# Autodesk Inventor assembly: Support
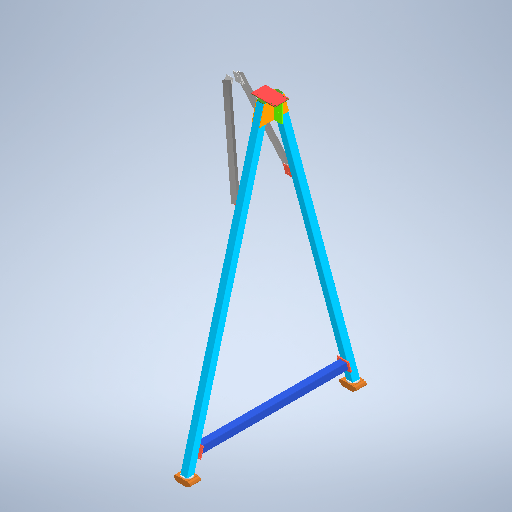
[picture p0: Inventor's stored thumbnail of the model, 512x512]
Saved by Autodesk Inventor 2025 (Build 290162010, 162A)
## iProperties
Created: 2024-06-18
Part Number: Support
Document SubType Name: Assembly
Designer: admin
Stock Number: Опора
Author: admin
## Documents named in this file (13)
- C:\Users\pokla\Documents\Inventor\Goat\Support.iam
- C:\Users\pokla\Documents\Inventor\Goat\Сrane plate 3.ipt
- C:\Users\pokla\Documents\Inventor\Goat\Stand.ipt
- C:\Users\pokla\Documents\Inventor\Goat\Сrane plate 4.ipt
- C:\Users\pokla\Documents\Inventor\Goat\Сrane plate 6.ipt
- C:\Users\pokla\Documents\Inventor\Goat\Сrane plate 2.ipt
- C:\Users\pokla\Documents\Inventor\Goat\Сrane plate 5.ipt
- C:\Users\pokla\Documents\Inventor\Goat\roller platform.ipt
- C:\Users\pokla\Documents\Inventor\Goat\foot.ipt
- C:\Users\pokla\Documents\Inventor\Goat\Crossbar.ipt
- C:\Users\pokla\Documents\Inventor\Goat\Сrane plate 1.ipt
- C:\Users\pokla\Documents\Inventor\Goat\Оттяжки.iam
- C:\Users\pokla\Documents\Inventor\Goat\Оттяжка 2.iam
## Components (24 placed, 12 different names)
1. Сrane plate 3.ipt:1 — Mate:11, Mate:12, Mate:13, Flush:6, Flush:7, Rigid:3
2. Stand.ipt:1 — Mate:9, Mate:10, Rigid:1
3. Сrane plate 4.ipt:1
4. Сrane plate 6.ipt:1 — Rigid:7
5. Сrane plate 4.ipt:2
6. Сrane plate 2.ipt:1 — Mate:11, Mate:12, Mate:13
7. Сrane plate 5.ipt:1 — Mate:9, Mate:10
8. roller platform.ipt:1 — Rigid:2, Mate:14
9. foot.ipt:1 — Rigid:1, Rigid:2
10. Сrane plate 3.ipt:2 — Rigid:3, Rigid:4, Mate:18, Mate:20
11. Сrane plate 2.ipt:2 — Rigid:4, Mate:19, Mate:21, Mate:23, Rigid:9
12. Сrane plate 4.ipt:3 — Mate:18, Mate:19, Flush:12, Flush:13
13. Сrane plate 4.ipt:4 — Mate:20, Mate:21, Mate:22, Mate:24
14. Stand.ipt:2 — Mate:23, Mate:24, Flush:13, Rigid:5, Mate:26, Mate:29, Flush:31, Mate:35, Mate:38
15. foot.ipt:2 — Rigid:5, Rigid:6
16. roller platform.ipt:2 — Rigid:6
17. Сrane plate 6.ipt:2 — Mate:26, Mate:27, Rigid:8, Mate:38
18. Сrane plate 5.ipt:3 — Mate:29, Flush:31, Mate:35
19. Сrane plate 6.ipt:3 — Rigid:7
20. Сrane plate 6.ipt:4 — Rigid:8, Mate:41
21. Crossbar.ipt:1 — Mate:39, Mate:40, Mate:41
22. Сrane plate 1:1 — Rigid:9
23. Оттяжки:1 [sub-assembly]
24. Оттяжка 2:1 [sub-assembly]
## Relationships (52: Mate 31, Flush 10, WeldJoint 9, RevoluteJoint 2)
- [Mate]: Stand.ipt:1 ↔ Сrane plate 4.ipt:1
- [Mate]: Stand.ipt:1 ↔ Сrane plate 4.ipt:2
- [Flush]: Stand.ipt:1 ↔ Сrane plate 4.ipt:2
- [Flush]: Stand.ipt:1 ↔ Сrane plate 4.ipt:1
- [Flush]: Stand.ipt:1 ↔ Сrane plate 4.ipt:1
- [Flush]: Stand.ipt:1 ↔ Сrane plate 4.ipt:2
- [Flush]: Stand.ipt:1 ↔ Сrane plate 2.ipt:1
- [Mate]: Stand.ipt:1 ↔ Сrane plate 2.ipt:1
- [Mate]: Stand.ipt:1 ↔ Сrane plate 6.ipt:1
- [Mate]: Stand.ipt:1 ↔ Сrane plate 6.ipt:1
- [Mate]: Сrane plate 3.ipt:1 ↔ Сrane plate 4.ipt:2
- [Mate] (-200 mm): Stand.ipt:1 ↔ Сrane plate 6.ipt:1
- [Mate]: Stand.ipt:1 ↔ Сrane plate 5.ipt:1
- Mate:9 (-45 mm): Stand.ipt:1 ↔ Сrane plate 5.ipt:1
- Mate:10 (1271 mm): Stand.ipt:1 ↔ Сrane plate 5.ipt:1
- Mate:11: Сrane plate 3.ipt:1 ↔ Сrane plate 2.ipt:1
- Mate:12: Сrane plate 3.ipt:1 ↔ Сrane plate 2.ipt:1
- Mate:13: Сrane plate 3.ipt:1 ↔ Сrane plate 2.ipt:1
- Flush:6: Сrane plate 3.ipt:1
- Flush:7: Сrane plate 3.ipt:1
- Rigid:1 [WeldJoint]: Stand.ipt:1 ↔ foot.ipt:1
- Rigid:2 [WeldJoint]: roller platform.ipt:1 ↔ foot.ipt:1
- Mate:14: roller platform.ipt:1
- [RevoluteJoint]: Сrane plate 5.ipt:1 ↔ Оттяжки:1
- Rigid:3 [WeldJoint]: Сrane plate 3.ipt:1 ↔ Сrane plate 3.ipt:2
- Rigid:4 [WeldJoint]: Сrane plate 3.ipt:2 ↔ Сrane plate 2.ipt:2
- Mate:18: Сrane plate 3.ipt:2 ↔ Сrane plate 4.ipt:3
- Mate:19: Сrane plate 2.ipt:2 ↔ Сrane plate 4.ipt:3
- Flush:12 (60 mm): Сrane plate 4.ipt:3
- Mate:20: Сrane plate 3.ipt:2 ↔ Сrane plate 4.ipt:4
- Mate:21: Сrane plate 2.ipt:2 ↔ Сrane plate 4.ipt:4
- Mate:22 (60 mm): Сrane plate 4.ipt:4
- Mate:23: Сrane plate 2.ipt:2 ↔ Stand.ipt:2
- Mate:24: Сrane plate 4.ipt:4 ↔ Stand.ipt:2
- Flush:13: Сrane plate 4.ipt:3 ↔ Stand.ipt:2
- Rigid:5 [WeldJoint]: Stand.ipt:2 ↔ foot.ipt:2
- Rigid:6 [WeldJoint]: foot.ipt:2 ↔ roller platform.ipt:2
- [Mate]: Сrane plate 5.ipt:1 ↔ Оттяжки:1
- Mate:26: Stand.ipt:2 ↔ Сrane plate 6.ipt:2
- Mate:27: Сrane plate 6.ipt:2
- Mate:29: Stand.ipt:2 ↔ Сrane plate 5.ipt:3
- Flush:31 (45 mm): Stand.ipt:2 ↔ Сrane plate 5.ipt:3
- Mate:35 (1271 mm): Stand.ipt:2 ↔ Сrane plate 5.ipt:3
- [RevoluteJoint]: Сrane plate 5.ipt:3 ↔ Оттяжка 2:1
- [Mate]: Сrane plate 5.ipt:3 ↔ Оттяжка 2:1
- Rigid:7 [WeldJoint]: Сrane plate 6.ipt:1 ↔ Сrane plate 6.ipt:3
- Rigid:8 [WeldJoint]: Сrane plate 6.ipt:2 ↔ Сrane plate 6.ipt:4
- Mate:38 (-200 mm): Stand.ipt:2 ↔ Сrane plate 6.ipt:2
- Mate:39: Crossbar.ipt:1
- Mate:40: Crossbar.ipt:1
- Mate:41 (26.8 mm): Сrane plate 6.ipt:4 ↔ Crossbar.ipt:1
- Rigid:9 [WeldJoint]: Сrane plate 2.ipt:2 ↔ Сrane plate 1:1
